# Autodesk Inventor assembly: Rueda
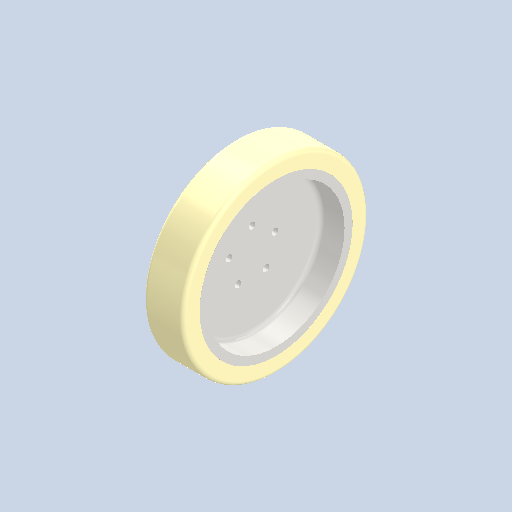
[picture p0: Inventor's stored thumbnail of the model, 512x512]
Saved by Autodesk Inventor 2022.1 (Build 261234000, 234)
## iProperties
Created: 2021-09-22
Part Number: Rueda
Document SubType Name: Assembly
Designer: seb_0
Author: seb_0
## Documents named in this file (3)
- C:\Users\seb_0\Desktop\PDM\ProyectoRobotPallet\Motor\Rueda\Rueda.iam
- C:\Users\seb_0\Desktop\PDM\ProyectoRobotPallet\Motor\Rueda\Interior_Rueda.ipt
- C:\Users\seb_0\Desktop\PDM\ProyectoRobotPallet\Motor\Rueda\Exterior_Rueda.ipt
## Components (2 placed, 2 different names)
1. Interior_Rueda:1 — Coincidencia:1, Coincidencia:2, Coincidencia:3, Nivelación:1, Coincidencia:4, Rotación:1
2. Exterior_Rueda:1 — Coincidencia:3, Nivelación:1, Rotación:1
## Relationships (6: Mate 4, Flush 1, RelateRotation 1)
- Coincidencia:1 [Mate]: Interior_Rueda:1
- Coincidencia:2 [Mate]: Interior_Rueda:1
- Coincidencia:3 [Mate]: Interior_Rueda:1 ↔ Exterior_Rueda:1
- Nivelación:1 [Flush]: Interior_Rueda:1 ↔ Exterior_Rueda:1
- Coincidencia:4 [Mate] (30 mm): Interior_Rueda:1
- Rotación:1 [RelateRotation] (1 ul): Interior_Rueda:1 ↔ Exterior_Rueda:1
